# Autodesk Inventor assembly: Ensamblaje2
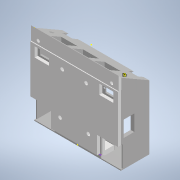
[picture p0: Inventor's stored thumbnail of the model, 180x180]
Saved by Autodesk Inventor 2021 (Build 250183000, 183)
## iProperties
Created: 2021-11-15
Part Number: Ensamblaje2
Document SubType Name: Weldment
Designer: Juan Camilo
Weld Material: Welded Aluminum-6061
Author: Juan Camilo
## Documents named in this file (5)
- C:\Users\Juan Camilo\OneDrive - Universidad de los Andes\Escritorio\Onixium\Ensamblaje2.iam
- C:\Users\Juan Camilo\OneDrive - Universidad de los Andes\Escritorio\Onixium\Base Onixium2.ipt
- C:\Users\Juan Camilo\OneDrive - Universidad de los Andes\Escritorio\Onixium\PlacaInferior.ipt
- C:\Users\Juan Camilo\OneDrive - Universidad de los Andes\Escritorio\Onixium\Cuchilla Versión 1.ipt
- C:\Users\Juan Camilo\OneDrive - Universidad de los Andes\Escritorio\Onixium\PiezaAtras.ipt
## Components (4 placed, 4 different names)
1. Base Onixium2:1 — Coincidencia:1, Coincidencia:2, Coincidencia:3
2. PlacaInferior:1 — Coincidencia:1
3. Cuchilla Versión 1:1 — Coincidencia:2
4. PiezaAtras:1 — Coincidencia:3
## Relationships (3: Mate 3)
- Coincidencia:1 [Mate]: Base Onixium2:1 ↔ PlacaInferior:1
- Coincidencia:2 [Mate]: Base Onixium2:1 ↔ Cuchilla Versión 1:1
- Coincidencia:3 [Mate]: Base Onixium2:1 ↔ PiezaAtras:1
